# Autodesk Inventor assembly: Simple Drawer
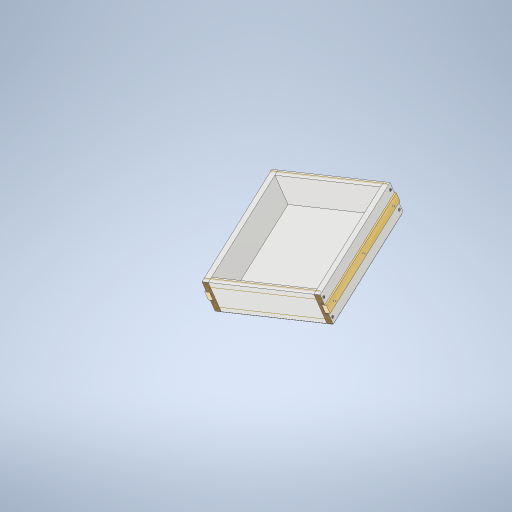
[picture p0: Inventor's stored thumbnail of the model, 512x512]
Saved by Autodesk Inventor 2024 (Build 280153000, 153)
## iProperties
RuleStatus: InUse
Category: Drawer
Created: 2023-03-30
Part Number: Simple Drawer
Document SubType Name: Assembly
Designer: sauliusd
Description: Simple Drawer
Author: sauliusd
## Documents named in this file (12)
- C:\W4INV 2024 Design\iBOX LIBRARY\Drawers\Simple Drawer\Simple Drawer.iam
- C:\W4INV 2024 Design\iBOX LIBRARY\Drawers\Simple Drawer\Parts\Drawer Front.ipt
- C:\W4INV 2024 Design\iBOX LIBRARY\Drawers\Simple Drawer\Parts\Drawer Back.ipt
- C:\W4INV 2024 Design\iBOX LIBRARY\Drawers\Simple Drawer\Parts\Drawer Bottom.ipt
- C:\W4INV 2024 Design\iBOX LIBRARY\Drawers\Simple Drawer\Parts\Drawer Left Side.ipt
- C:\W4INV 2024 Design\iBOX LIBRARY\Drawers\Simple Drawer\Parts\Drawer Right Side.ipt
- C:\W4INV 2024 Design\iBOX LIBRARY\Drawers\Simple Drawer\Parts\Drawer Left Runner.ipt
- C:\W4INV 2024 Design\iBOX LIBRARY\Drawers\Simple Drawer\Parts\Drawer Right Runner.ipt
- C:\W4INV 2024 Design\_LIBRARY\Fixed joints\Screws\WOOD SCREW CROSS RECESSED FLAT HEAD\Wood screw Cross Recessed Flat Head M3.5x25 H.ipt
- C:\W4INV 2024 Design\iBOX LIBRARY\Drawers\Simple Drawer\Parts\Drawer Skeleton.ipt
- C:\W4INV 2023 Design\LIBRARY\Fixed joints\Screws\WOOD SCREW CROSS RECESSED FLAT HEAD.ipt
- C:\W4INV 2024 Design\_LIBRARY\Fixed joints\Screws\WOOD SCREW CROSS RECESSED FLAT HEAD\Wood screw Cross Recessed Flat Head M4.5x70 H.ipt
## Components (22 placed, 10 different names)
1. @Skeleton — Flush:1, Flush:2, Flush:3
2. Drawer Front:1 — Flush:4, Flush:5, First Axis Plane:1, First Axis Plane:2, Second Axis Plane:5, Second Axis Plane:6
3. Drawer Back:1 — First Axis Plane:3, First Axis Plane:4, Second Axis Plane:7, Second Axis Plane:8
4. Drawer Bottom:1
5. Drawer Left Side:1 — Screw plane surface:1, Screw plane surface:2, Screw plane surface:3, Screw plane surface:4
6. Drawer Right Side:1 — Screw plane surface:5, Screw plane surface:6, Screw plane surface:7, Screw plane surface:8
7. Drawer Left Runner:1 — Insert:1
8. Drawer Right Runner:1 — Insert:2
9. Wood screw Cross Recessed Flat Head M4.5x70 H:11 — Second Axis Plane:1, Screw plane surface:1, First Axis Plane:1
10. Wood screw Cross Recessed Flat Head M4.5x70 H:12 — Second Axis Plane:2, Screw plane surface:2, First Axis Plane:2
11. Wood screw Cross Recessed Flat Head M4.5x70 H:13 — Second Axis Plane:3, Screw plane surface:3, First Axis Plane:3
12. Wood screw Cross Recessed Flat Head M4.5x70 H:14 — Second Axis Plane:4, Screw plane surface:4, First Axis Plane:4
13. Wood screw Cross Recessed Flat Head M4.5x70 H:16 — Second Axis Plane:5, First Axis Plane:5, Screw plane surface:5
14. Wood screw Cross Recessed Flat Head M4.5x70 H:17 — Second Axis Plane:6, First Axis Plane:6, Screw plane surface:6
15. Wood screw Cross Recessed Flat Head M4.5x70 H:18 — Second Axis Plane:7, First Axis Plane:7, Screw plane surface:7
16. Wood screw Cross Recessed Flat Head M4.5x70 H:19 — Second Axis Plane:8, First Axis Plane:8, Screw plane surface:8
17. Wood screw Cross Recessed Flat Head M3.5x25 H:2 — Insert:2
18. Wood screw Cross Recessed Flat Head M3.5x25 H:3
19. Wood screw Cross Recessed Flat Head M3.5x25 H:4
20. Wood screw Cross Recessed Flat Head M3.5x25 H:1 — Insert:1
21. Wood screw Cross Recessed Flat Head M3.5x25 H:8
22. Wood screw Cross Recessed Flat Head M3.5x25 H:9
## Component patterns: (3 elements, first: Wood screw Cross Recessed Flat Head M3.5x25 H:2), (3 elements, first: Wood screw Cross Recessed Flat Head M3.5x25 H:1)
## Relationships (31: Mate 16, Flush 13, Insert 2)
- Insert:1: Drawer Left Runner:1 ↔ Wood screw Cross Recessed Flat Head M3.5x25 H:1
- Insert:2: Drawer Right Runner:1 ↔ Wood screw Cross Recessed Flat Head M3.5x25 H:2
- Flush:1: @Skeleton
- Flush:2: @Skeleton
- Flush:3: @Skeleton
- Flush:4 (-16 mm): Drawer Front:1
- Flush:5 (-16 mm): Drawer Front:1
- Second Axis Plane:1 [Mate]: Wood screw Cross Recessed Flat Head M4.5x70 H:11
- Screw plane surface:1 [Flush]: Drawer Left Side:1 ↔ Wood screw Cross Recessed Flat Head M4.5x70 H:11
- First Axis Plane:1 [Mate]: Drawer Front:1 ↔ Wood screw Cross Recessed Flat Head M4.5x70 H:11
- Second Axis Plane:2 [Mate]: Wood screw Cross Recessed Flat Head M4.5x70 H:12
- Screw plane surface:2 [Flush]: Drawer Left Side:1 ↔ Wood screw Cross Recessed Flat Head M4.5x70 H:12
- First Axis Plane:2 [Mate]: Drawer Front:1 ↔ Wood screw Cross Recessed Flat Head M4.5x70 H:12
- Second Axis Plane:3 [Mate]: Wood screw Cross Recessed Flat Head M4.5x70 H:13
- Screw plane surface:3 [Flush]: Drawer Left Side:1 ↔ Wood screw Cross Recessed Flat Head M4.5x70 H:13
- First Axis Plane:3 [Mate]: Drawer Back:1 ↔ Wood screw Cross Recessed Flat Head M4.5x70 H:13
- Second Axis Plane:4 [Mate]: Wood screw Cross Recessed Flat Head M4.5x70 H:14
- Screw plane surface:4 [Flush]: Drawer Left Side:1 ↔ Wood screw Cross Recessed Flat Head M4.5x70 H:14
- First Axis Plane:4 [Mate]: Drawer Back:1 ↔ Wood screw Cross Recessed Flat Head M4.5x70 H:14
- Second Axis Plane:5 [Mate]: Drawer Front:1 ↔ Wood screw Cross Recessed Flat Head M4.5x70 H:16
- First Axis Plane:5 [Mate]: Wood screw Cross Recessed Flat Head M4.5x70 H:16
- Screw plane surface:5 [Flush]: Drawer Right Side:1 ↔ Wood screw Cross Recessed Flat Head M4.5x70 H:16
- Second Axis Plane:6 [Mate]: Drawer Front:1 ↔ Wood screw Cross Recessed Flat Head M4.5x70 H:17
- First Axis Plane:6 [Mate]: Wood screw Cross Recessed Flat Head M4.5x70 H:17
- Screw plane surface:6 [Flush]: Drawer Right Side:1 ↔ Wood screw Cross Recessed Flat Head M4.5x70 H:17
- Second Axis Plane:7 [Mate]: Drawer Back:1 ↔ Wood screw Cross Recessed Flat Head M4.5x70 H:18
- First Axis Plane:7 [Mate]: Wood screw Cross Recessed Flat Head M4.5x70 H:18
- Screw plane surface:7 [Flush]: Drawer Right Side:1 ↔ Wood screw Cross Recessed Flat Head M4.5x70 H:18
- Second Axis Plane:8 [Mate]: Drawer Back:1 ↔ Wood screw Cross Recessed Flat Head M4.5x70 H:19
- First Axis Plane:8 [Mate]: Wood screw Cross Recessed Flat Head M4.5x70 H:19
- Screw plane surface:8 [Flush]: Drawer Right Side:1 ↔ Wood screw Cross Recessed Flat Head M4.5x70 H:19
## Named parameters: BoardT = 18 mm, Inlet = 0 mm, RearSpace = 10 mm
